# Autodesk Inventor assembly: AM14U2_Long
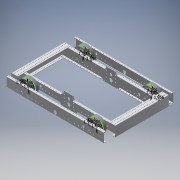
[picture p0: Inventor's stored thumbnail of the model, 180x180]
Saved by Autodesk Inventor 2016 (Build 200138000, 138)
## iProperties
Category: Drive Base
Company: Autodesk Inc.
Created: 2014-12-16
Part Number: AM14U2_Long
Document SubType Name: Assembly
Designer: Autodesk Inc.
Catalog Web Link: andymark.com
Vendor: Andy Mark Inc.
Author: Autodesk Inc.
## Documents named in this file (2)
- C:\Users\Administrator\Desktop\3192CAD\InitialRobotProto\DB_DriveBaseLong_AM14U2.iam
- C:\Users\Administrator\Desktop\3192CAD\InitialRobotProto\amparts\AM14U2 Half Long.iam
## Components (2 placed, 2 different names)
1. AM14U2 Half Long_1 [sub-assembly] — Insert:1, Insert:2, Mate:1, Mate:2, Mate:3
2. AM14U2 Half Long_2 [sub-assembly] — Insert:1, Insert:2, Mate:1, Mate:2, Mate:3
## Relationships (5: Mate 3, Insert 2)
- Insert:1: AM14U2 Half Long_1 ↔ AM14U2 Half Long_2
- Insert:2: AM14U2 Half Long_1 ↔ AM14U2 Half Long_2
- Mate:1: AM14U2 Half Long_1 ↔ AM14U2 Half Long_2
- Mate:2: AM14U2 Half Long_1 ↔ AM14U2 Half Long_2
- Mate:3: AM14U2 Half Long_1 ↔ AM14U2 Half Long_2
